# Autodesk Inventor assembly: rcache
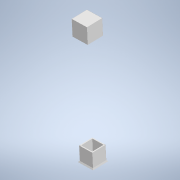
[picture p0: Inventor's stored thumbnail of the model, 180x180]
Saved by Autodesk Inventor 2021 (Build 250183000, 183)
## iProperties
Created: 2020-06-13
Part Number: rcache
Document SubType Name: Assembly
Designer: Yatekii
Author: Yatekii
## Documents named in this file (3)
- C:\Users\Yatekii\repos\rcache\rcache.iam
- C:\Users\Yatekii\repos\rcache\inner.iam
- C:\Users\Yatekii\repos\rcache\outer.iam
## Components (2 placed, 2 different names)
1. inner:1 [sub-assembly] — Slider:1
2. outer:1 [sub-assembly] — Slider:1
## Relationships (1: TranslationJoint 1)
- Slider:1 [TranslationJoint]: inner:1 ↔ outer:1
